# Autodesk Inventor assembly: force_sensor_v2
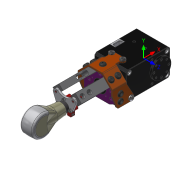
[picture p0: Inventor's stored thumbnail of the model, 180x180]
Saved by Autodesk Inventor 2019.4 (Build 234330000, 330)
## iProperties
Created: 2018-02-01
Part Number: force_sensor_v2
Material: 一般
Document SubType Name: Assembly
Designer: y6tada
Mass: 98.3533 g
Surface Area: 375.997 cm^2
Volume: 64.3806 cm^3
Density: 1.52768 g/cm^3
Author: y6tada
## Documents named in this file (23)
- C:\Workspace\HaptHexa\Hardware\Inventor\Tibia\_Tibia.iam
- C:\Workspace\HaptHexa\Hardware\Inventor\Tibia\leg_pipe_cfrp.ipt
- C:\Workspace\HaptHexa\Hardware\Inventor\X430\XL-430.iam
- C:\Workspace\HaptHexa\Hardware\Inventor\Tibia\plate.ipt
- C:\Workspace\HaptHexa\Hardware\Inventor\Tibia\load_cell_v2.ipt
- C:\Workspace\HaptHexa\Hardware\Inventor\Tibia\lod_holder.ipt
- C:\Workspace\HaptHexa\Hardware\Inventor\Tibia\con_sensor_lod.ipt
- C:\Workspace\HaptHexa\Hardware\Inventor\Tibia\z_sensor_base.ipt
- C:\Workspace\HaptHexa\Hardware\Inventor\Tibia\lod_base.ipt
- C:\Workspace\HaptHexa\Hardware\Inventor\Tibia\pin_2x15.ipt
- C:\Workspace\HaptHexa\Hardware\Inventor\Tibia\force_sensor_pcb_assy.iam
- C:\Workspace\HaptHexa\Hardware\Inventor\Tibia\SHOE_ASM.iam
- C:\Users\y6tada\Documents\Inventor\Content Center Files\R2019\ja-JP\ISO 4762(2)\ISO 4762 - M1.6 x 10ISO.ipt
- C:\Users\y6tada\Documents\Inventor\Content Center Files\R2019\ja-JP\ISO 7380-1\ISO 7380-1 - M3 x 6.ipt
- C:\Users\y6tada\Documents\Inventor\Content Center Files\R2019\ja-JP\JIS B 1111(1)\JIS B 1111 - M2.5x5(1).ipt
- C:\Users\y6tada\Documents\Inventor\Content Center Files\R2019\ja-JP\JIS B 1111(1)\JIS B 1111 - M2.5x14(1).ipt
- C:\Users\y6tada\Documents\Inventor\Content Center Files\R2019\ja-JP\JIS B 1176\JIS B 1176 - M1.6 x 6 - 0.35.ipt
- D:\2019.3 - HaptHexa\Hardware\Mech\Inventor\Tibia\_Tibia\AIP\FEA\csifsck2o.fins
- D:\2019.3 - HaptHexa\Hardware\Mech\Inventor\Tibia\_Tibia\AIP\FEA\csifsck2o.fsat
- D:\2019.3 - HaptHexa\Hardware\Mech\Inventor\Tibia\_Tibia\AIP\FEA\csifsck2o.ftes
- D:\2019.3 - HaptHexa\Hardware\Mech\Inventor\Tibia\_Tibia\AIP\FEA\csifsck2o.fwiz
- D:\2019.3 - HaptHexa\Hardware\Mech\Inventor\Tibia\_Tibia\AIP\FEA\csifsck9s.fmsh
- D:\2019.3 - HaptHexa\Hardware\Mech\Inventor\Tibia\_Tibia\AIP\FEA\csifsck9t.fres
## Components (30 placed, 16 different names)
1. XL-430:1 [sub-assembly] — メイト:29, メイト:30, メイト:31, メイト:43, フラッシュ:8, メイト:60, フラッシュ:9
2. leg_pipe_cfrp:1 — メイト:40, メイト:41, メイト:46, メイト:47, メイト:59, メイト:61, メイト:62, フラッシュ:64, メイト:63
3. plate:1 — メイト:29, メイト:30, メイト:31, メイト:34, メイト:35, メイト:36, メイト:37, メイト:38, メイト:39, メイト:48, メイト:49, 挿入:2, 挿入:3, 挿入:4, 挿入:5, 挿入:6, 挿入:7, 挿入:8, 挿入:9, 挿入:10, 挿入:11, 挿入:12, 挿入:13, 挿入:14
4. load_cell_v2:1 — メイト:34, メイト:35, メイト:36, フラッシュ:1, メイト:55, フラッシュ:4
5. load_cell_v2:2 — メイト:37, メイト:38, メイト:39, メイト:56, フラッシュ:5
6. lod_holder:1 — メイト:40, フラッシュ:1, フラッシュ:2, メイト:42, 挿入:1, メイト:62
7. con_sensor_lod:1 — フラッシュ:2, メイト:41, メイト:42, 挿入:15, 挿入:16, 挿入:17
8. z_sensor_base:1 — メイト:43, メイト:48, メイト:49, メイト:50, メイト:51, メイト:53, メイト:57, メイト:58, 角度:3
9. lod_base:1 — メイト:46, メイト:47, メイト:50, メイト:51, メイト:53
10. pin_2x15:1 — メイト:55, フラッシュ:4
11. pin_2x15:2 — メイト:56, フラッシュ:5
12. force_sensor_pcb_assy:1 [sub-assembly] — メイト:57, メイト:58, 角度:3
13. SHOE_ASM:1 [sub-assembly] — メイト:59, メイト:61, メイト:63
14. ISO 4762 M1.6 x 10:1 — 挿入:1
15. ISO 7380-1 M3 x 6:1 — 挿入:2
16. ISO 7380-1 M3 x 6:2 — 挿入:3
17. ISO 7380-1 M3 x 6:3 — 挿入:4
18. ISO 7380-1 M3 x 6:4 — 挿入:5
19. ISO 7380-1 M3 x 6:5 — 挿入:6
20. ISO 7380-1 M3 x 6:6 — 挿入:7
21. ISO 7380-1 M3 x 6:7 — 挿入:8
22. ISO 7380-1 M3 x 6:8 — 挿入:9
23. ISO 7380-1 M3 x 6:9 — 挿入:10
24. JIS B 1111 M2.5x5:1 — 挿入:11
25. JIS B 1111 M2.5x5:2 — 挿入:12
26. JIS B 1111 M2.5x14:1 — 挿入:13
27. JIS B 1111 M2.5x14:2 — 挿入:14
28. JIS B 1176 - メートル M1.6 x 6:1 — 挿入:15
29. JIS B 1176 - メートル M1.6 x 6:2 — 挿入:16
30. JIS B 1176 - メートル M1.6 x 6:3 — 挿入:17
## Relationships (54: Mate 29, Insert 17, Flush 7, Angle 1)
- メイト:29 [Mate]: XL-430:1 ↔ plate:1
- メイト:30 [Mate]: XL-430:1 ↔ plate:1
- メイト:31 [Mate]: XL-430:1 ↔ plate:1
- メイト:34 [Mate]: plate:1 ↔ load_cell_v2:1
- メイト:35 [Mate]: plate:1 ↔ load_cell_v2:1
- メイト:36 [Mate]: plate:1 ↔ load_cell_v2:1
- メイト:37 [Mate]: plate:1 ↔ load_cell_v2:2
- メイト:38 [Mate]: plate:1 ↔ load_cell_v2:2
- メイト:39 [Mate]: plate:1 ↔ load_cell_v2:2
- メイト:40 [Mate]: leg_pipe_cfrp:1 ↔ lod_holder:1
- フラッシュ:1 [Flush] (-1 mm): load_cell_v2:1 ↔ lod_holder:1
- フラッシュ:2 [Flush]: lod_holder:1 ↔ con_sensor_lod:1
- メイト:41 [Mate]: leg_pipe_cfrp:1 ↔ con_sensor_lod:1
- メイト:42 [Mate]: lod_holder:1 ↔ con_sensor_lod:1
- メイト:43 [Mate] (3 mm): XL-430:1 ↔ z_sensor_base:1
- メイト:46 [Mate]: leg_pipe_cfrp:1 ↔ lod_base:1
- メイト:47 [Mate]: leg_pipe_cfrp:1 ↔ lod_base:1
- メイト:48 [Mate]: plate:1 ↔ z_sensor_base:1
- メイト:49 [Mate]: plate:1 ↔ z_sensor_base:1
- メイト:50 [Mate]: z_sensor_base:1 ↔ lod_base:1
- メイト:51 [Mate]: z_sensor_base:1 ↔ lod_base:1
- メイト:53 [Mate]: z_sensor_base:1 ↔ lod_base:1
- メイト:55 [Mate]: load_cell_v2:1 ↔ pin_2x15:1
- フラッシュ:4 [Flush] (3 mm): load_cell_v2:1 ↔ pin_2x15:1
- メイト:56 [Mate]: load_cell_v2:2 ↔ pin_2x15:2
- フラッシュ:5 [Flush] (3 mm): load_cell_v2:2 ↔ pin_2x15:2
- メイト:57 [Mate]: z_sensor_base:1 ↔ force_sensor_pcb_assy:1
- メイト:58 [Mate]: z_sensor_base:1 ↔ force_sensor_pcb_assy:1
- 角度:3 [Angle] (0 deg): z_sensor_base:1 ↔ force_sensor_pcb_assy:1
- メイト:59 [Mate]: leg_pipe_cfrp:1 ↔ SHOE_ASM:1
- 挿入:1 [Insert]: lod_holder:1 ↔ ISO 4762 M1.6 x 10:1
- 挿入:2 [Insert]: plate:1 ↔ ISO 7380-1 M3 x 6:1
- 挿入:3 [Insert]: plate:1 ↔ ISO 7380-1 M3 x 6:2
- 挿入:4 [Insert]: plate:1 ↔ ISO 7380-1 M3 x 6:3
- 挿入:5 [Insert]: plate:1 ↔ ISO 7380-1 M3 x 6:4
- 挿入:6 [Insert]: plate:1 ↔ ISO 7380-1 M3 x 6:5
- 挿入:7 [Insert]: plate:1 ↔ ISO 7380-1 M3 x 6:6
- 挿入:8 [Insert]: plate:1 ↔ ISO 7380-1 M3 x 6:7
- 挿入:9 [Insert]: plate:1 ↔ ISO 7380-1 M3 x 6:8
- 挿入:10 [Insert]: plate:1 ↔ ISO 7380-1 M3 x 6:9
- 挿入:11 [Insert]: plate:1 ↔ JIS B 1111 M2.5x5:1
- 挿入:12 [Insert]: plate:1 ↔ JIS B 1111 M2.5x5:2
- 挿入:13 [Insert]: plate:1 ↔ JIS B 1111 M2.5x14:1
- 挿入:14 [Insert]: plate:1 ↔ JIS B 1111 M2.5x14:2
- 挿入:15 [Insert]: con_sensor_lod:1 ↔ JIS B 1176 - メートル M1.6 x 6:1
- 挿入:16 [Insert]: con_sensor_lod:1 ↔ JIS B 1176 - メートル M1.6 x 6:2
- 挿入:17 [Insert]: con_sensor_lod:1 ↔ JIS B 1176 - メートル M1.6 x 6:3
- フラッシュ:8 [Flush]: XL-430:1
- メイト:60 [Mate]: XL-430:1
- フラッシュ:9 [Flush]: XL-430:1
- メイト:61 [Mate]: leg_pipe_cfrp:1 ↔ SHOE_ASM:1
- メイト:62 [Mate]: leg_pipe_cfrp:1 ↔ lod_holder:1
- フラッシュ:64 [Flush]: leg_pipe_cfrp:1
- メイト:63 [Mate]: leg_pipe_cfrp:1 ↔ SHOE_ASM:1
## Named parameters: sa_0 = 1e-13, sa_1 = -6e-13, sa_2 = -500, sa_3 = -353.553, sa_4 = -5e-13, sa_5 = -353.553, sa_6 = -500, sa_7 = -0, sa_8 = -1e-13, sa_9 = -0, sa_10 = 500, sa_11 = -6e-13
note: some values were not read from the file. Shown as the stored number, unit unknown: "sa_0", "sa_1", "sa_2", "sa_3", "sa_4", "sa_5", "sa_6", "sa_7", "sa_8", "sa_9", "sa_10", "sa_11".
